# Autodesk Inventor assembly: Assembly1
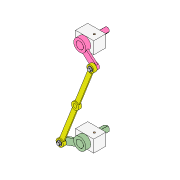
[picture p0: Inventor's stored thumbnail of the model, 180x180]
Saved by Autodesk Inventor 2017 (Build 210142000, 142)
## iProperties
Created: 2020-07-24
Part Number: Assembly1
Document SubType Name: Assembly
Designer: admin
Author: admin
## Documents named in this file (6)
- F:\YouTube\2021\YouTube\9S\17SixLinkReverser\Assembly2test.iam
- F:\YouTube\2021\YouTube\9S\17SixLinkReverser\Bearing.ipt
- F:\YouTube\2021\YouTube\9S\17SixLinkReverser\Crank1.ipt
- F:\YouTube\2021\YouTube\9S\17SixLinkReverser\Conrod3.ipt
- F:\YouTube\2021\YouTube\9S\17SixLinkReverser\Pin.ipt
- F:\YouTube\2021\YouTube\9S\17SixLinkReverser\Bolt3W.ipt
## Components (9 placed, 5 different names)
1. Pin:1 — Insert:7
2. Pin:2 — Insert:8
3. Bearing:2 — Flush:1, Flush:2, Flush:3, Insert:2, Insert:8
4. Bearing:1 — Flush:1, Flush:2, Flush:3, Insert:6, Insert:7
5. Crank1:3 — Insert:3, Insert:6, Insert:12
6. Crank1:2 — Insert:2, Insert:10, Insert:13
7. Conrod3:1 — Insert:3, Insert:13
8. Bolt3W:1 — Insert:12
9. Bolt3W:3 — Insert:10
## Relationships (11: Insert 8, Flush 3)
- Flush:1: Bearing:2 ↔ Bearing:1
- Flush:2: Bearing:2 ↔ Bearing:1
- Flush:3 (-140 mm): Bearing:2 ↔ Bearing:1
- Insert:2: Bearing:2 ↔ Crank1:2
- Insert:3: Crank1:3 ↔ Conrod3:1
- Insert:6: Bearing:1 ↔ Crank1:3
- Insert:7: Pin:1 ↔ Bearing:1
- Insert:8: Pin:2 ↔ Bearing:2
- Insert:10: Crank1:2 ↔ Bolt3W:3
- Insert:12: Crank1:3 ↔ Bolt3W:1
- Insert:13: Crank1:2 ↔ Conrod3:1
